# Autodesk Inventor assembly: Timing_Assy
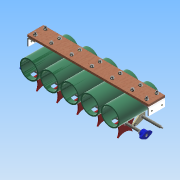
[picture p0: Inventor's stored thumbnail of the model, 180x180]
Saved by Autodesk Inventor 2018.1 (Build 221171000, 171)
## iProperties
Created: 2019-02-11
Part Number: Timing_Assy
Document SubType Name: Assembly
Designer: James
Author: James
## Documents named in this file (16)
- C:\Users\admin\Desktop\Ball Sorting Machine\Ball-Sorting-Machine\Timing Gate\Timing_Assy.iam
- C:\Users\admin\Desktop\Ball Sorting Machine\Ball-Sorting-Machine\Timing Gate\PVC Pipe.ipt
- C:\Users\admin\Desktop\Ball Sorting Machine\Ball-Sorting-Machine\Timing Gate\Timing_Star.ipt
- C:\Users\admin\Desktop\Ball Sorting Machine\Ball-Sorting-Machine\Timing Gate\Timing_Lever.ipt
- C:\Users\admin\Desktop\Ball Sorting Machine\Ball-Sorting-Machine\Timing Gate\Timing_Lever Weight.ipt
- C:\Users\admin\Desktop\Ball Sorting Machine\Ball-Sorting-Machine\Timing Gate\BS 3673 - 6mm External Circlip.ipt
- C:\Users\admin\Desktop\Ball Sorting Machine\Ball-Sorting-Machine\Timing Gate\M3 x 0.5mm Zinc Plated Steel Washer.ipt
- C:\Users\admin\Desktop\Ball Sorting Machine\Ball-Sorting-Machine\Timing Gate\Socket Button Head - (A2) - M3 x 10.ipt
- C:\Users\admin\Desktop\Ball Sorting Machine\Ball-Sorting-Machine\Timing Gate\Timing_Lever Shaft.ipt
- C:\Users\admin\Desktop\Ball Sorting Machine\Ball-Sorting-Machine\Timing Gate\Timing_Star Shaft.ipt
- C:\Users\admin\Desktop\Ball Sorting Machine\Ball-Sorting-Machine\Timing Gate\Timing_Backboard.ipt
- C:\Users\admin\Desktop\Ball Sorting Machine\Ball-Sorting-Machine\Timing Gate\Nyloc Nut - M4.ipt
- C:\Users\admin\Desktop\Ball Sorting Machine\Ball-Sorting-Machine\Timing Gate\Socket Csk Screw - (A2) - M4 x  16.ipt
- C:\Users\admin\Desktop\Ball Sorting Machine\Ball-Sorting-Machine\Timing Gate\SAFL212 Oval 2 Bolt Flanged Unit.ipt
- C:\Users\admin\Desktop\Ball Sorting Machine\Ball-Sorting-Machine\Timing Gate\Timing_Angle Bracket.ipt
- C:\Users\admin\Desktop\Ball Sorting Machine\Ball-Sorting-Machine\Timing Gate\Socket Cap Screw - Standard - (A2) - M4 x 16.ipt
## Components (82 placed, 15 different names)
1. Timing_Backboard:1 — Flush:18, Mate:51, Mate:52, Mate:53, Tangent:1, Flush:19, Flush:20, Mate:55, Mate:56, Mate:59, Mate:60, Flush:22, Flush:23, Mate:67, Mate:68, Mate:69, Flush:27, Flush:28, Mate:74, Mate:75, Flush:29, Mate:82, Flush:30, Mate:83, Mate:84, Mate:85
2. Timing_Star Shaft:1 — Mate:4, Flush:6, Flush:14, Flush:15, Mate:49, Mate:50, Angle:3, Mate:61, Mate:62, Mate:63, Mate:66
3. Timing_Lever:1 — Flush:7, Mate:6, Mate:7, Mate:8, Flush:9, Mate:13, Mate:14, Mate:16
4. Timing_Lever Shaft:1 — Flush:8, Mate:6, Flush:9, Mate:9, Mate:10, Mate:11, Mate:12, Mate:41, Mate:42, Mate:43, Mate:44, Flush:16, Flush:17
5. Timing_Lever Weight:1 — Mate:7, Mate:8
6. M3 x 0.5mm Zinc Plated Steel Washer:1 — Mate:13, Mate:14, Mate:15
7. Socket Button Head - (A2) - M3 x 10:1 — Mate:15, Mate:16
8. Timing_Lever:2 — Mate:41, Mate:48
9. Timing_Lever Weight:2
10. M3 x 0.5mm Zinc Plated Steel Washer:2
11. Socket Button Head - (A2) - M3 x 10:2
12. Timing_Lever:3 — Mate:42, Mate:47
13. Timing_Lever Weight:3
14. M3 x 0.5mm Zinc Plated Steel Washer:3
15. Socket Button Head - (A2) - M3 x 10:3
16. Timing_Lever:4 — Mate:43, Mate:46
17. Timing_Lever Weight:4
18. M3 x 0.5mm Zinc Plated Steel Washer:4
19. Socket Button Head - (A2) - M3 x 10:4
20. Timing_Lever:5 — Mate:44, Mate:45
21. Timing_Lever Weight:5
22. M3 x 0.5mm Zinc Plated Steel Washer:5
23. Socket Button Head - (A2) - M3 x 10:5
24. SAFL212 Oval 2 Bolt Flanged Unit:1 — Flush:22, Mate:61, Flush:24, Angle:4, Mate:65
25. SAFL212 Oval 2 Bolt Flanged Unit:2 — Mate:62, Flush:23, Flush:24, Mate:64
26. BS 3673 - 6mm External Circlip:16 — Mate:65, Mate:66, Flush:25
27. BS 3673 - 6mm External Circlip:17 — Mate:63, Mate:64, Flush:25, Flush:26
28. Timing_Angle Bracket:1 — Mate:67, Mate:68, Mate:69, Flush:27, Flush:28, Mate:70, Mate:71, Mate:72, Mate:73
29. Nyloc Nut - M4:13 — Mate:74, Mate:76
30. Socket Cap Screw - Standard - (A2) - M4 x 16:3 — Mate:72, Mate:73, Mate:77
31. Nyloc Nut - M4:14 — Mate:75, Mate:77
32. Socket Cap Screw - Standard - (A2) - M4 x 16:4 — Mate:70, Mate:71, Mate:76
33. Timing_Angle Bracket:2 — Flush:29, Mate:82, Flush:30, Mate:83
34. Socket Cap Screw - Standard - (A2) - M4 x 16:5 — Mate:87
35. Socket Cap Screw - Standard - (A2) - M4 x 16:6 — Mate:86
36. Nyloc Nut - M4:15 — Mate:84, Mate:87
37. Nyloc Nut - M4:16 — Mate:85, Mate:86
38. PVC Pipe:1 — Angle:1, Mate:5, Flush:7, Mate:51, Mate:52, Tangent:1, Mate:54
39. Nyloc Nut - M4:1 — Mate:58, Mate:59
40. Socket Csk Screw - (A2) - M4 x  16:1 — Mate:54, Mate:55, Flush:21, Mate:57
41. Socket Csk Screw - (A2) - M4 x  16:2 — Flush:21, Mate:56, Mate:58
42. Nyloc Nut - M4:2 — Mate:57, Mate:60
43. PVC Pipe:2
44. Nyloc Nut - M4:3
45. Socket Csk Screw - (A2) - M4 x  16:3
46. Socket Csk Screw - (A2) - M4 x  16:7
47. Nyloc Nut - M4:7
48. PVC Pipe:3
49. Nyloc Nut - M4:4
50. Socket Csk Screw - (A2) - M4 x  16:4
51. Socket Csk Screw - (A2) - M4 x  16:8
52. Nyloc Nut - M4:8
53. PVC Pipe:4
54. Nyloc Nut - M4:5
55. Socket Csk Screw - (A2) - M4 x  16:5
56. Socket Csk Screw - (A2) - M4 x  16:9
57. Nyloc Nut - M4:9
58. PVC Pipe:5 — Mate:53
59. Nyloc Nut - M4:6
60. Socket Csk Screw - (A2) - M4 x  16:6
61. Socket Csk Screw - (A2) - M4 x  16:10
62. Nyloc Nut - M4:10
63. BS 3673 - 6mm External Circlip:2 — Mate:9, Mate:12, Flush:10, Angle:2
64. BS 3673 - 6mm External Circlip:1 — Mate:10, Mate:11, Flush:10
65. BS 3673 - 6mm External Circlip:3 — Mate:48
66. BS 3673 - 6mm External Circlip:4
67. BS 3673 - 6mm External Circlip:5 — Mate:47
68. BS 3673 - 6mm External Circlip:6
69. BS 3673 - 6mm External Circlip:7 — Mate:46
70. BS 3673 - 6mm External Circlip:8
71. BS 3673 - 6mm External Circlip:9 — Mate:45
72. BS 3673 - 6mm External Circlip:10
73. BS 3673 - 6mm External Circlip:11 — Mate:49, Mate:50, Angle:3, Flush:26
74. Timing_Star:1 — Mate:4, Mate:5
75. BS 3673 - 6mm External Circlip:12
76. Timing_Star:2
77. BS 3673 - 6mm External Circlip:13
78. Timing_Star:3
79. BS 3673 - 6mm External Circlip:14
80. Timing_Star:4
81. BS 3673 - 6mm External Circlip:15
82. Timing_Star:5
## Component patterns: (5 elements, first: PVC Pipe:1 + Nyloc Nut - M4:1 + Socket Csk Screw - (A2) - M4 x  16:1 + Socket Csk Screw - (A2) - M4 x  16:2 + Nyloc Nut - M4:2), (5 elements, first: BS 3673 - 6mm External Circlip:2 + BS 3673 - 6mm External Circlip:1), (5 elements, first: BS 3673 - 6mm External Circlip:11 + Timing_Star:1)
## Relationships (114: Mate 84, Flush 25, Angle 4, Tangent 1)
- Angle:1 (180 deg): PVC Pipe:1
- Mate:4: Timing_Star Shaft:1 ↔ Timing_Star:1
- Mate:5 (1 mm): PVC Pipe:1 ↔ Timing_Star:1
- Flush:6: Timing_Star Shaft:1
- Flush:7 (1 mm): Timing_Lever:1 ↔ PVC Pipe:1
- Flush:8: Timing_Lever Shaft:1
- Mate:6: Timing_Lever:1 ↔ Timing_Lever Shaft:1
- Mate:7: Timing_Lever:1 ↔ Timing_Lever Weight:1
- Mate:8: Timing_Lever:1 ↔ Timing_Lever Weight:1
- Flush:9: Timing_Lever:1 ↔ Timing_Lever Shaft:1
- Mate:9: Timing_Lever Shaft:1 ↔ BS 3673 - 6mm External Circlip:2
- Mate:10: Timing_Lever Shaft:1 ↔ BS 3673 - 6mm External Circlip:1
- Mate:11: Timing_Lever Shaft:1 ↔ BS 3673 - 6mm External Circlip:1
- Mate:12: Timing_Lever Shaft:1 ↔ BS 3673 - 6mm External Circlip:2
- Flush:10: BS 3673 - 6mm External Circlip:2 ↔ BS 3673 - 6mm External Circlip:1
- Angle:2 (180 deg): BS 3673 - 6mm External Circlip:2
- Mate:13: Timing_Lever:1 ↔ M3 x 0.5mm Zinc Plated Steel Washer:1
- Mate:14: Timing_Lever:1 ↔ M3 x 0.5mm Zinc Plated Steel Washer:1
- Mate:15: M3 x 0.5mm Zinc Plated Steel Washer:1 ↔ Socket Button Head - (A2) - M3 x 10:1
- Mate:16: Timing_Lever:1 ↔ Socket Button Head - (A2) - M3 x 10:1
- [Mate]: Timing_Lever:2 ↔ Timing_Lever Weight:2
- [Mate]: Timing_Lever:2 ↔ Timing_Lever Weight:2
- [Mate]: Timing_Lever:2 ↔ M3 x 0.5mm Zinc Plated Steel Washer:2
- [Mate]: Timing_Lever:2 ↔ M3 x 0.5mm Zinc Plated Steel Washer:2
- [Mate]: M3 x 0.5mm Zinc Plated Steel Washer:2 ↔ Socket Button Head - (A2) - M3 x 10:2
- [Mate]: Timing_Lever:2 ↔ Socket Button Head - (A2) - M3 x 10:2
- [Mate]: Timing_Lever:3 ↔ Timing_Lever Weight:3
- [Mate]: Timing_Lever:3 ↔ Timing_Lever Weight:3
- [Mate]: Timing_Lever:3 ↔ M3 x 0.5mm Zinc Plated Steel Washer:3
- [Mate]: Timing_Lever:3 ↔ M3 x 0.5mm Zinc Plated Steel Washer:3
- [Mate]: M3 x 0.5mm Zinc Plated Steel Washer:3 ↔ Socket Button Head - (A2) - M3 x 10:3
- [Mate]: Timing_Lever:3 ↔ Socket Button Head - (A2) - M3 x 10:3
- [Mate]: Timing_Lever:4 ↔ Timing_Lever Weight:4
- [Mate]: Timing_Lever:4 ↔ Timing_Lever Weight:4
- [Mate]: Timing_Lever:4 ↔ M3 x 0.5mm Zinc Plated Steel Washer:4
- [Mate]: Timing_Lever:4 ↔ M3 x 0.5mm Zinc Plated Steel Washer:4
- [Mate]: M3 x 0.5mm Zinc Plated Steel Washer:4 ↔ Socket Button Head - (A2) - M3 x 10:4
- [Mate]: Timing_Lever:4 ↔ Socket Button Head - (A2) - M3 x 10:4
- [Mate]: Timing_Lever:5 ↔ Timing_Lever Weight:5
- [Mate]: Timing_Lever:5 ↔ Timing_Lever Weight:5
- [Mate]: Timing_Lever:5 ↔ M3 x 0.5mm Zinc Plated Steel Washer:5
- [Mate]: Timing_Lever:5 ↔ M3 x 0.5mm Zinc Plated Steel Washer:5
- [Mate]: M3 x 0.5mm Zinc Plated Steel Washer:5 ↔ Socket Button Head - (A2) - M3 x 10:5
- [Mate]: Timing_Lever:5 ↔ Socket Button Head - (A2) - M3 x 10:5
- Mate:41: Timing_Lever Shaft:1 ↔ Timing_Lever:2
- Mate:42: Timing_Lever Shaft:1 ↔ Timing_Lever:3
- Mate:43: Timing_Lever Shaft:1 ↔ Timing_Lever:4
- Mate:44: Timing_Lever Shaft:1 ↔ Timing_Lever:5
- Mate:45: Timing_Lever:5 ↔ BS 3673 - 6mm External Circlip:9
- Mate:46: Timing_Lever:4 ↔ BS 3673 - 6mm External Circlip:7
- Mate:47: Timing_Lever:3 ↔ BS 3673 - 6mm External Circlip:5
- Mate:48: Timing_Lever:2 ↔ BS 3673 - 6mm External Circlip:3
- Flush:11 (-58 mm)
- Flush:12 (-5 mm)
- Flush:13 (30 mm)
- Flush:14: Timing_Star Shaft:1
- Flush:15: Timing_Star Shaft:1
- Flush:16: Timing_Lever Shaft:1
- Flush:17: Timing_Lever Shaft:1
- Mate:49: Timing_Star Shaft:1 ↔ BS 3673 - 6mm External Circlip:11
- Mate:50: Timing_Star Shaft:1 ↔ BS 3673 - 6mm External Circlip:11
- Angle:3 (0 deg): Timing_Star Shaft:1 ↔ BS 3673 - 6mm External Circlip:11
- Flush:18: Timing_Backboard:1
- Mate:51: Timing_Backboard:1 ↔ PVC Pipe:1
- Mate:52: Timing_Backboard:1 ↔ PVC Pipe:1
- Mate:53: Timing_Backboard:1 ↔ PVC Pipe:5
- Tangent:1: Timing_Backboard:1 ↔ PVC Pipe:1
- Flush:19: Timing_Backboard:1
- Flush:20: Timing_Backboard:1
- Mate:54: PVC Pipe:1 ↔ Socket Csk Screw - (A2) - M4 x  16:1
- Mate:55 (-10.3 mm): Timing_Backboard:1 ↔ Socket Csk Screw - (A2) - M4 x  16:1
- Flush:21: Socket Csk Screw - (A2) - M4 x  16:1 ↔ Socket Csk Screw - (A2) - M4 x  16:2
- Mate:56: Timing_Backboard:1 ↔ Socket Csk Screw - (A2) - M4 x  16:2
- Mate:57: Socket Csk Screw - (A2) - M4 x  16:1 ↔ Nyloc Nut - M4:2
- Mate:58: Nyloc Nut - M4:1 ↔ Socket Csk Screw - (A2) - M4 x  16:2
- Mate:59: Timing_Backboard:1 ↔ Nyloc Nut - M4:1
- Mate:60: Timing_Backboard:1 ↔ Nyloc Nut - M4:2
- Flush:22: Timing_Backboard:1 ↔ SAFL212 Oval 2 Bolt Flanged Unit:1
- Mate:61: Timing_Star Shaft:1 ↔ SAFL212 Oval 2 Bolt Flanged Unit:1
- Mate:62: Timing_Star Shaft:1 ↔ SAFL212 Oval 2 Bolt Flanged Unit:2
- Flush:23: Timing_Backboard:1 ↔ SAFL212 Oval 2 Bolt Flanged Unit:2
- Flush:24: SAFL212 Oval 2 Bolt Flanged Unit:1 ↔ SAFL212 Oval 2 Bolt Flanged Unit:2
- Angle:4 (0 deg): SAFL212 Oval 2 Bolt Flanged Unit:1
- Mate:63: Timing_Star Shaft:1 ↔ BS 3673 - 6mm External Circlip:17
- Mate:64: SAFL212 Oval 2 Bolt Flanged Unit:2 ↔ BS 3673 - 6mm External Circlip:17
- Mate:65: SAFL212 Oval 2 Bolt Flanged Unit:1 ↔ BS 3673 - 6mm External Circlip:16
- Mate:66: Timing_Star Shaft:1 ↔ BS 3673 - 6mm External Circlip:16
- Flush:25: BS 3673 - 6mm External Circlip:16 ↔ BS 3673 - 6mm External Circlip:17
- Flush:26: BS 3673 - 6mm External Circlip:17 ↔ BS 3673 - 6mm External Circlip:11
- Mate:67: Timing_Backboard:1 ↔ Timing_Angle Bracket:1
- Mate:68: Timing_Backboard:1 ↔ Timing_Angle Bracket:1
- Mate:69: Timing_Backboard:1 ↔ Timing_Angle Bracket:1
- Flush:27: Timing_Backboard:1 ↔ Timing_Angle Bracket:1
- Flush:28: Timing_Backboard:1 ↔ Timing_Angle Bracket:1
- Mate:70: Timing_Angle Bracket:1 ↔ Socket Cap Screw - Standard - (A2) - M4 x 16:4
- Mate:71: Timing_Angle Bracket:1 ↔ Socket Cap Screw - Standard - (A2) - M4 x 16:4
- Mate:72: Timing_Angle Bracket:1 ↔ Socket Cap Screw - Standard - (A2) - M4 x 16:3
- Mate:73: Timing_Angle Bracket:1 ↔ Socket Cap Screw - Standard - (A2) - M4 x 16:3
- Mate:74: Timing_Backboard:1 ↔ Nyloc Nut - M4:13
- Mate:75: Timing_Backboard:1 ↔ Nyloc Nut - M4:14
- Mate:76: Nyloc Nut - M4:13 ↔ Socket Cap Screw - Standard - (A2) - M4 x 16:4
- Mate:77: Socket Cap Screw - Standard - (A2) - M4 x 16:3 ↔ Nyloc Nut - M4:14
- [Mate]: Timing_Angle Bracket:2 ↔ Socket Cap Screw - Standard - (A2) - M4 x 16:6
- [Mate]: Timing_Angle Bracket:2 ↔ Socket Cap Screw - Standard - (A2) - M4 x 16:6
- [Mate]: Timing_Angle Bracket:2 ↔ Socket Cap Screw - Standard - (A2) - M4 x 16:5
- [Mate]: Timing_Angle Bracket:2 ↔ Socket Cap Screw - Standard - (A2) - M4 x 16:5
- Flush:29: Timing_Backboard:1 ↔ Timing_Angle Bracket:2
- Mate:82: Timing_Backboard:1 ↔ Timing_Angle Bracket:2
- Flush:30: Timing_Backboard:1 ↔ Timing_Angle Bracket:2
- Mate:83: Timing_Backboard:1 ↔ Timing_Angle Bracket:2
- Mate:84: Timing_Backboard:1 ↔ Nyloc Nut - M4:15
- Mate:85: Timing_Backboard:1 ↔ Nyloc Nut - M4:16
- Mate:86: Socket Cap Screw - Standard - (A2) - M4 x 16:6 ↔ Nyloc Nut - M4:16
- Mate:87: Socket Cap Screw - Standard - (A2) - M4 x 16:5 ↔ Nyloc Nut - M4:15
## Named parameters: d37_d20 = 0 mm, d38_d21 = 0 mm, d39_d33 = 0 mm, d40_d34 = 0 mm, d41_d35 = 0 mm, d42_d36 = 0 mm, d43_d20 = 0 mm, d44_d21 = 0 mm, d45_d33 = 0 mm, d46_d34 = 0 mm, d47_d35 = 0 mm, d48_d36 = 0 mm, d49_d20 = 0 mm, d50_d21 = 0 mm, d51_d33 = 0 mm, d52_d34 = 0 mm, d53_d35 = 0 mm, d54_d36 = 0 mm, d55_d20 = 0 mm, d56_d21 = 0 mm, d57_d33 = 0 mm, d58_d34 = 0 mm, d59_d35 = 0 mm, d60_d36 = 0 mm, d139_d131 = 0 mm, d140_d132 = 0 mm, d141_d133 = 0 mm, d142_d134 = 0 mm
